# Autodesk Inventor assembly: TR1 Actuator
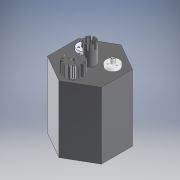
[picture p0: Inventor's stored thumbnail of the model, 180x180]
Saved by Autodesk Inventor 2017 (Build 210142000, 142)
## iProperties
Created: 2018-10-09
Part Number: TR1 Actuator
Document SubType Name: Assembly
Designer: Zach
Author: Zach
## Documents named in this file (13)
- C:\Users\Dell\Documents\GitHub\tr2\Arm Actuator\Arm Actuator.iam
- C:\Users\Dell\Documents\GitHub\tr2\Arm Actuator\TA01.ipt
- C:\Users\Dell\Documents\GitHub\tr2\Arm Actuator\TA02.ipt
- C:\Users\Dell\Documents\GitHub\tr2\Arm Actuator\Arm Actuator\Design Accelerator\Spur Gears2.iam
- C:\Users\Dell\Documents\GitHub\tr2\Arm Actuator\Arm Actuator\Design Accelerator\Spur Gears3.iam
- C:\Users\Dell\Documents\GitHub\tr2\Arm Actuator\TA03.ipt
- C:\Users\Dell\Documents\GitHub\tr2\Arm Actuator\EMS22XXX-D28-LSX.ipt
- C:\Users\Dell\Documents\GitHub\tr2\Arm Actuator\12RPM Gear Motor.ipt
- C:\Users\Dell\Documents\GitHub\tr2\Arm Actuator\Slip Ring.ipt
- C:\Users\Dell\Documents\GitHub\tr2\Arm Actuator\TA06.ipt
- C:\Users\Dell\Documents\GitHub\tr2\Arm Actuator\Bourns ACE 128.ipt
- C:\Users\Dell\Documents\GitHub\tr2\Arm Actuator\Thrust Bearing.ipt
- C:\Users\Dell\Documents\GitHub\tr2\Arm Actuator\6mm Mounting Hub, thin.ipt
## Components (16 placed, 11 different names)
1. TA01:1 — Mate:28, Mate:29, Mate:30
2. TA02:1 — Mate:2, Mate:3, Mate:4, Mate:5, Mate:6, Mate:7, Mate:16, Angle:1, Mate:20, Mate:21, Mate:22, Mate:24, Mate:28, Mate:29, Mate:30, Flush:1, Mate:38, Angle:2, Mate:39, Mate:40, Mate:43, Mate:46, Mate:48, Mate:50
3. TA03:1 — Mate:7, Mate:26, Mate:42, Mate:44
4. TA06:1 — Mate:34, Mate:35, Mate:36
5. Spur Gears:1 [sub-assembly] — Mate:2, Mate:26, Flush:1, Mate:31, Mate:32, Mate:33, Mate:36, Mate:44
6. Spur Gears:2 [sub-assembly] — Mate:3, Mate:4, Mate:51
7. Spur Gears:3 [sub-assembly] — Mate:5, Mate:6
8. Spur Gears:4 [sub-assembly] — Mate:23, Mate:24
9. Thrust Bearing:1 — Mate:42, Mate:43
10. 12RPM Gear Motor:1 — Mate:20, Mate:21, Mate:22, Mate:47
11. EMS22XXX-D28-LSX:1 — Mate:16, Angle:1, Mate:23, Mate:40, Mate:45
12. Bourns ACE 128:1 — Mate:38, Angle:2, Mate:39, Mate:49
13. Slip Ring:1 — Mate:31, Mate:32, Mate:33, Mate:34, Mate:35
14. 6mm Mounting Hub, thin:1 — Mate:45, Mate:46
15. 6mm Mounting Hub, thin:2 — Mate:47, Mate:48, Mate:51
16. 6mm Mounting Hub, thin:3 — Mate:49, Mate:50
## Relationships (38: Mate 35, Angle 2, Flush 1)
- Mate:2: TA02:1 ↔ Spur Gears:1
- Mate:3: TA02:1 ↔ Spur Gears:2
- Mate:4: TA02:1 ↔ Spur Gears:2
- Mate:5: TA02:1 ↔ Spur Gears:3
- Mate:6: TA02:1 ↔ Spur Gears:3
- Mate:7: TA02:1 ↔ TA03:1
- Mate:16: TA02:1 ↔ EMS22XXX-D28-LSX:1
- Angle:1 (0 deg): TA02:1 ↔ EMS22XXX-D28-LSX:1
- Mate:20: TA02:1 ↔ 12RPM Gear Motor:1
- Mate:21: TA02:1 ↔ 12RPM Gear Motor:1
- Mate:22: TA02:1 ↔ 12RPM Gear Motor:1
- Mate:23: Spur Gears:4 ↔ EMS22XXX-D28-LSX:1
- Mate:24: TA02:1 ↔ Spur Gears:4
- Mate:26: TA03:1 ↔ Spur Gears:1
- Mate:28: TA01:1 ↔ TA02:1
- Mate:29: TA01:1 ↔ TA02:1
- Mate:30: TA01:1 ↔ TA02:1
- Flush:1: TA02:1 ↔ Spur Gears:1
- Mate:31: Spur Gears:1 ↔ Slip Ring:1
- Mate:32: Spur Gears:1 ↔ Slip Ring:1
- Mate:33: Spur Gears:1 ↔ Slip Ring:1
- Mate:34: TA06:1 ↔ Slip Ring:1
- Mate:35: TA06:1 ↔ Slip Ring:1
- Mate:36: TA06:1 ↔ Spur Gears:1
- Mate:38: TA02:1 ↔ Bourns ACE 128:1
- Angle:2 (0 deg): TA02:1 ↔ Bourns ACE 128:1
- Mate:39: TA02:1 ↔ Bourns ACE 128:1
- Mate:40: TA02:1 ↔ EMS22XXX-D28-LSX:1
- Mate:42: TA03:1 ↔ Thrust Bearing:1
- Mate:43: TA02:1 ↔ Thrust Bearing:1
- Mate:44: TA03:1 ↔ Spur Gears:1
- Mate:45: EMS22XXX-D28-LSX:1 ↔ 6mm Mounting Hub, thin:1
- Mate:46: TA02:1 ↔ 6mm Mounting Hub, thin:1
- Mate:47: 12RPM Gear Motor:1 ↔ 6mm Mounting Hub, thin:2
- Mate:48: TA02:1 ↔ 6mm Mounting Hub, thin:2
- Mate:49: Bourns ACE 128:1 ↔ 6mm Mounting Hub, thin:3
- Mate:50: TA02:1 ↔ 6mm Mounting Hub, thin:3
- Mate:51: Spur Gears:2 ↔ 6mm Mounting Hub, thin:2
